# Autodesk Inventor assembly: Base
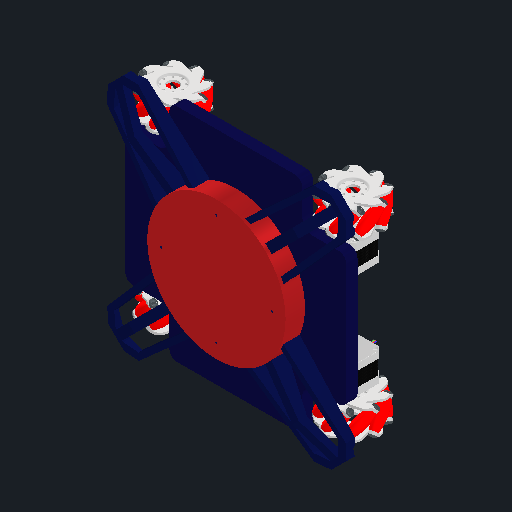
[picture p0: Inventor's stored thumbnail of the model, 512x512]
Saved by Autodesk Inventor 2023 (Build 270158000, 158)
## iProperties
Created: 2023-04-06
Part Number: Base
Document SubType Name: Assembly
Designer: vatdu
Author: vatdu
## Documents named in this file (6)
- C:\Users\vatdu\Desktop\CRYSTAL MARK II\Base Chassis\Base.iam
- C:\Users\vatdu\Desktop\CRYSTAL MARK II\Base Chassis\Base Motor.ipt
- C:\Users\vatdu\Desktop\CRYSTAL MARK II\Base Chassis\Wheels Cover.ipt
- C:\Users\vatdu\Desktop\CRYSTAL MARK II\Wheels\Mecanum Wheel.iam
- C:\Users\vatdu\Desktop\CRYSTAL MARK II\Components\Stepper Motor.ipt
- C:\Users\vatdu\Desktop\CRYSTAL MARK II\Base Chassis\Central Support.ipt
## Components (11 placed, 5 different names)
1. Base Motor:1 — Rotational:1, Rotational:2
2. Wheels Cover:1
3. Mecanum Wheel:1 [sub-assembly]
4. Mecanum Wheel:2 [sub-assembly]
5. Mecanum Wheel:3 [sub-assembly]
6. Mecanum Wheel:4 [sub-assembly]
7. Stepper Motor:1
8. Stepper Motor:2
9. Stepper Motor:3
10. Stepper Motor:4
11. Central Support:1 — Rotational:1, Rotational:2
## Relationships (2: RevoluteJoint 2)
- Rotational:1 [RevoluteJoint]: Base Motor:1 ↔ Central Support:1
- Rotational:2 [RevoluteJoint]: Base Motor:1 ↔ Central Support:1
